# Autodesk Inventor assembly: Assembly4
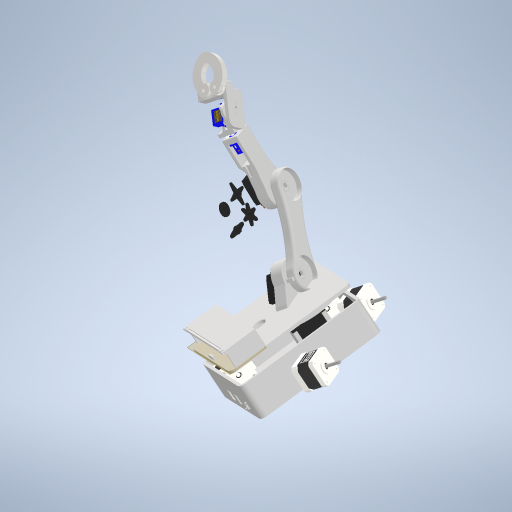
[picture p0: Inventor's stored thumbnail of the model, 512x512]
Saved by Autodesk Inventor 2024 (Build 280153000, 153)
## iProperties
Created: 2023-08-29
Part Number: Assembly4
Document SubType Name: Assembly
Designer: jebes windows
Author: jebes windows
## Documents named in this file (16)
- C:\Users\jebes windows\Documents\Inventor\Robotska_roka\Assembly4.iam
- C:\Users\jebes windows\Documents\Inventor\Robotska_roka\miza.ipt
- C:\Users\jebes windows\Documents\Inventor\Robotska_roka\servo-motor-mg996r-1.snapshot.1(2)\Servo Motor MG996R  With Attachments\Servo Motor MG996R  With Attachments.iam
- C:\Users\jebes windows\Documents\Inventor\Robotska_roka\roka1.ipt
- C:\Users\jebes windows\Documents\Inventor\Robotska_roka\roka2.ipt
- C:\Users\jebes windows\Documents\Inventor\Robotska_roka\sg90-micro-servo-9g-tower-pro-1.snapshot.3\SG90 - Micro Servo 9g - Tower Pro\SG90 - Micro Servo 9g - Tower Pro.iam
- C:\Users\jebes windows\Documents\Inventor\Robotska_roka\roka3.ipt
- C:\Users\jebes windows\Documents\Inventor\Robotska_roka\KLESCE.ipt
- C:\Users\jebes windows\Documents\Inventor\Robotska_roka\klesce2.ipt
- C:\Users\jebes windows\Documents\Inventor\Robotska_roka\Assembly4\Design Accelerator\Spur Gears2.iam
- C:\Users\jebes windows\Documents\Inventor\Robotska_roka\vozicek1.ipt
- C:\Users\jebes windows\Documents\Inventor\Robotska_roka\pokrow.ipt
- C:\Users\jebes windows\Documents\Inventor\Robotska_roka\Nema 17 Motor a Pasos 17HS4401\Nema 17 Motor a Pasos 17HS4401.ipt
- C:\Users\jebes windows\Documents\Inventor\Robotska_roka\ArduinoMega_STEP_AP203\ArduinoMega_STEP_AP203.ipt
- C:\Users\jebes windows\Documents\Inventor\Robotska_roka\pokrow2.ipt
- C:\Users\jebes windows\Documents\Inventor\Robotska_roka\zatic.ipt
## Components (25 placed, 15 different names)
1. Servo Motor MG996R  With Attachments:1 [sub-assembly] — Rotational:3, Flush:7
2. Servo Motor MG996R  With Attachments:2 [sub-assembly] — Rotational:3, Rotational:4
3. Servo Motor MG996R  With Attachments:3 [sub-assembly] — Rotational:5, Rigid:2
4. Servo Motor MG996R  With Attachments:4 [sub-assembly] — Rotational:5, Rotational:6
5. miza:1 — Rotational:4, Rigid:2
6. roka1:1 — Rotational:6, Rotational:8
7. Servo Motor MG996R  With Attachments:5 [sub-assembly] — Rigid:3
8. Servo Motor MG996R  With Attachments:6 [sub-assembly] — Rotational:8
9. roka2:1 — Rigid:3, Rotational:9
10. SG90 - Micro Servo 9g - Tower Pro:1 [sub-assembly] — Rotational:9, Flush:1, Flush:2
11. roka3:1 — Flush:1, Flush:2, Rotational:10
12. SG90 - Micro Servo 9g - Tower Pro:2 [sub-assembly] — Rotational:10, Flush:3, Flush:4
13. SG90 - Micro Servo 9g - Tower Pro:3 [sub-assembly] — Rotational:11, Rotational:12, Flush:5
14. KLESCE:1 — Flush:3, Flush:4, Rotational:11, Rotational:13
15. klesce2:1
16. Spur Gears:1 [sub-assembly] — Rotational:12, Flush:5, Rotational:13
17. vozicek1:1 — Flush:7, Rotational:14, Rigid:4, Rotational:15
18. pokrow:1 — Rotational:16, Flush:8, Flush:9
19. Nema 17 Motor a Pasos 17HS4401:1 — Rotational:14
20. Nema 17 Motor a Pasos 17HS4401:2
21. Nema 17 Motor a Pasos 17HS4401:3 — Rigid:4
22. Nema 17 Motor a Pasos 17HS4401:4
23. ArduinoMega_STEP_AP203:1 — Rotational:15
24. pokrow2:1 — Rotational:16
25. zatic:1 — Flush:8, Flush:9
## Relationships (25: RevoluteJoint 14, Flush 8, WeldJoint 3)
- Rotational:3 [RevoluteJoint]: Servo Motor MG996R  With Attachments:1 ↔ Servo Motor MG996R  With Attachments:2
- Rotational:4 [RevoluteJoint]: Servo Motor MG996R  With Attachments:2 ↔ miza:1
- Rotational:5 [RevoluteJoint]: Servo Motor MG996R  With Attachments:3 ↔ Servo Motor MG996R  With Attachments:4
- Rigid:2 [WeldJoint]: Servo Motor MG996R  With Attachments:3 ↔ miza:1
- Rotational:6 [RevoluteJoint]: Servo Motor MG996R  With Attachments:4 ↔ roka1:1
- [RevoluteJoint]: Servo Motor MG996R  With Attachments:5 ↔ Servo Motor MG996R  With Attachments:6
- Rotational:8 [RevoluteJoint]: roka1:1 ↔ Servo Motor MG996R  With Attachments:6
- Rigid:3 [WeldJoint]: Servo Motor MG996R  With Attachments:5 ↔ roka2:1
- Rotational:9 [RevoluteJoint]: roka2:1 ↔ SG90 - Micro Servo 9g - Tower Pro:1
- Flush:1: SG90 - Micro Servo 9g - Tower Pro:1 ↔ roka3:1
- Flush:2: SG90 - Micro Servo 9g - Tower Pro:1 ↔ roka3:1
- Rotational:10 [RevoluteJoint]: roka3:1 ↔ SG90 - Micro Servo 9g - Tower Pro:2
- Flush:3: SG90 - Micro Servo 9g - Tower Pro:2 ↔ KLESCE:1
- Flush:4: SG90 - Micro Servo 9g - Tower Pro:2 ↔ KLESCE:1
- Rotational:11 [RevoluteJoint]: SG90 - Micro Servo 9g - Tower Pro:3 ↔ KLESCE:1
- Rotational:12 [RevoluteJoint]: SG90 - Micro Servo 9g - Tower Pro:3 ↔ Spur Gears:1
- Flush:5: SG90 - Micro Servo 9g - Tower Pro:3 ↔ Spur Gears:1
- Rotational:13 [RevoluteJoint]: KLESCE:1 ↔ Spur Gears:1
- Flush:7: Servo Motor MG996R  With Attachments:1 ↔ vozicek1:1
- Rotational:14 [RevoluteJoint]: vozicek1:1 ↔ Nema 17 Motor a Pasos 17HS4401:1
- Rigid:4 [WeldJoint]: vozicek1:1 ↔ Nema 17 Motor a Pasos 17HS4401:3
- Rotational:15 [RevoluteJoint]: vozicek1:1 ↔ ArduinoMega_STEP_AP203:1
- Rotational:16 [RevoluteJoint]: pokrow:1 ↔ pokrow2:1
- Flush:8: pokrow:1 ↔ zatic:1
- Flush:9: pokrow:1 ↔ zatic:1
## Named parameters: d42_d35 = 0 mm, d43_d36 = -21.582819 deg
